# Autodesk Inventor assembly: Diseño Piezas
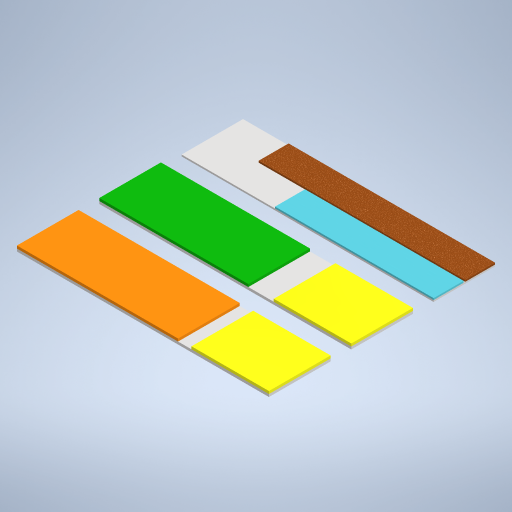
[picture p0: Inventor's stored thumbnail of the model, 512x512]
Saved by Autodesk Inventor 2024 (Build 280153000, 153)
## iProperties
Created: 2023-07-08
Part Number: Diseño Piezas
Document SubType Name: Assembly
Designer: sergi
Author: sergi
## Documents named in this file (8)
- C:\Users\sergi\OneDrive\Escritorio\Piso\Escritorio Piso\Escritorio2\Diseño Piezas.iam
- C:\Users\sergi\OneDrive\Escritorio\Piso\Escritorio Piso\Escritorio2\Tabla Grande 1.ipt
- C:\Users\sergi\OneDrive\Escritorio\Piso\Escritorio Piso\Escritorio2\PataMadera1.ipt
- C:\Users\sergi\OneDrive\Escritorio\Piso\Escritorio Piso\Escritorio2\Tapa 1.ipt
- C:\Users\sergi\OneDrive\Escritorio\Piso\Escritorio Piso\Escritorio2\Tapa 2.ipt
- C:\Users\sergi\OneDrive\Escritorio\Piso\Escritorio Piso\Escritorio2\Tabla fina.ipt
- C:\Users\sergi\OneDrive\Escritorio\Piso\Escritorio Piso\Escritorio2\Madera Inferior 2.ipt
- C:\Users\sergi\OneDrive\Escritorio\Piso\Escritorio Piso\Escritorio2\Madera Inferior1.ipt
## Components (9 placed, 7 different names)
1. Tabla Grande 1:1 — Nivelación:1, Coincidencia:1, Nivelación:2, Coincidencia:4, Nivelación:5, Nivelación:6, Nivelación:7, Coincidencia:5, Nivelación:8, Nivelación:11, Coincidencia:7, Nivelación:12
2. PataMadera1:1 — Coincidencia:4, Nivelación:5, Nivelación:6
3. PataMadera1:2 — Coincidencia:3, Nivelación:3, Nivelación:4
4. Tabla Grande 1:2 — Nivelación:1, Coincidencia:1, Nivelación:2, Coincidencia:3, Nivelación:3, Nivelación:4, Nivelación:9, Coincidencia:6, Nivelación:10
5. Tapa 1:1 — Nivelación:9, Coincidencia:6, Nivelación:10
6. Tapa 2:1 — Nivelación:7, Coincidencia:5, Nivelación:8
7. Tabla fina:1 — Nivelación:11, Coincidencia:7, Nivelación:12, Coincidencia:8, Nivelación:13, Nivelación:14, Coincidencia:9, Nivelación:15, Nivelación:16
8. Madera Inferior 2:1 — Coincidencia:9, Nivelación:15, Nivelación:16
9. Madera Inferior1:1 — Coincidencia:8, Nivelación:13, Nivelación:14
## Relationships (24: Flush 16, Mate 8)
- Nivelación:1 [Flush]: Tabla Grande 1:1 ↔ Tabla Grande 1:2
- Coincidencia:1 [Mate] (200 mm): Tabla Grande 1:1 ↔ Tabla Grande 1:2
- Nivelación:2 [Flush]: Tabla Grande 1:1 ↔ Tabla Grande 1:2
- Coincidencia:3 [Mate]: PataMadera1:2 ↔ Tabla Grande 1:2
- Nivelación:3 [Flush]: PataMadera1:2 ↔ Tabla Grande 1:2
- Nivelación:4 [Flush]: PataMadera1:2 ↔ Tabla Grande 1:2
- Coincidencia:4 [Mate]: Tabla Grande 1:1 ↔ PataMadera1:1
- Nivelación:5 [Flush]: Tabla Grande 1:1 ↔ PataMadera1:1
- Nivelación:6 [Flush]: Tabla Grande 1:1 ↔ PataMadera1:1
- Nivelación:7 [Flush]: Tabla Grande 1:1 ↔ Tapa 2:1
- Coincidencia:5 [Mate]: Tabla Grande 1:1 ↔ Tapa 2:1
- Nivelación:8 [Flush]: Tabla Grande 1:1 ↔ Tapa 2:1
- Nivelación:9 [Flush]: Tabla Grande 1:2 ↔ Tapa 1:1
- Coincidencia:6 [Mate]: Tabla Grande 1:2 ↔ Tapa 1:1
- Nivelación:10 [Flush]: Tabla Grande 1:2 ↔ Tapa 1:1
- Nivelación:11 [Flush]: Tabla Grande 1:1 ↔ Tabla fina:1
- Coincidencia:7 [Mate] (200 mm): Tabla Grande 1:1 ↔ Tabla fina:1
- Nivelación:12 [Flush]: Tabla Grande 1:1 ↔ Tabla fina:1
- Coincidencia:8 [Mate]: Tabla fina:1 ↔ Madera Inferior1:1
- Nivelación:13 [Flush]: Tabla fina:1 ↔ Madera Inferior1:1
- Nivelación:14 [Flush]: Tabla fina:1 ↔ Madera Inferior1:1
- Coincidencia:9 [Mate]: Tabla fina:1 ↔ Madera Inferior 2:1
- Nivelación:15 [Flush]: Tabla fina:1 ↔ Madera Inferior 2:1
- Nivelación:16 [Flush]: Tabla fina:1 ↔ Madera Inferior 2:1
